# Autodesk Inventor assembly: ArmWithBase
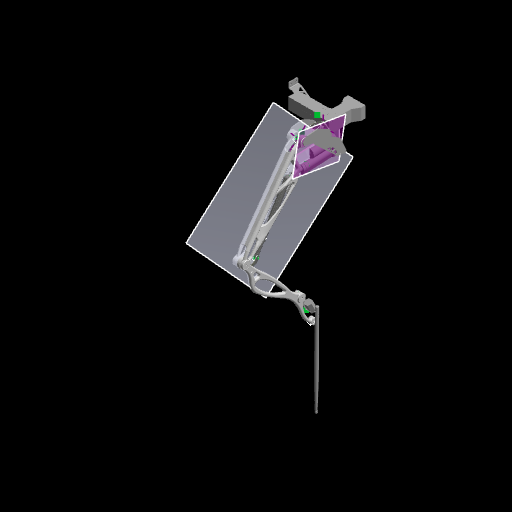
[picture p0: Inventor's stored thumbnail of the model, 512x512]
Saved by Autodesk Inventor 2025.2 (Build 292293000, 293)
## iProperties
Created: 2025-01-19
Part Number: ArmWithBase
Document SubType Name: Assembly
Designer: valer
Author: valer
## Documents named in this file (5)
- C:\Users\valer\Desktop\str1ker\cad\ArmFrontLeft.iam
- C:\Users\valer\Desktop\str1ker\cad\ArmBase.iam
- C:\Users\valer\Desktop\str1ker\cad\Arm.iam
- C:\Users\valer\Desktop\str1ker\cad\ArmScapula.ipt
- C:\Users\valer\Desktop\str1ker\cad\ArmScapulaMirror.ipt
## Components (4 placed, 4 different names)
1. Base:1 [sub-assembly] — Mate:5, Mate:6, Mate:7, Mate:9, Mate:10, Mate:11, Mate:12
2. Arm:1 [sub-assembly] — Mate:5, Mate:6, Mate:8
3. ArmScapula:1 — Mate:9
4. ArmScapulaMirror:1 — Mate:10, Mate:11, Mate:12
## Relationships (8: Mate 8)
- Mate:5: Base:1 ↔ Arm:1
- Mate:6: Base:1 ↔ Arm:1
- Mate:7: Base:1
- Mate:8: Arm:1
- Mate:9: Base:1 ↔ ArmScapula:1
- Mate:10: Base:1 ↔ ArmScapulaMirror:1
- Mate:11: Base:1 ↔ ArmScapulaMirror:1
- Mate:12: Base:1 ↔ ArmScapulaMirror:1
